# Autodesk Inventor assembly: 18659_pack_assembly
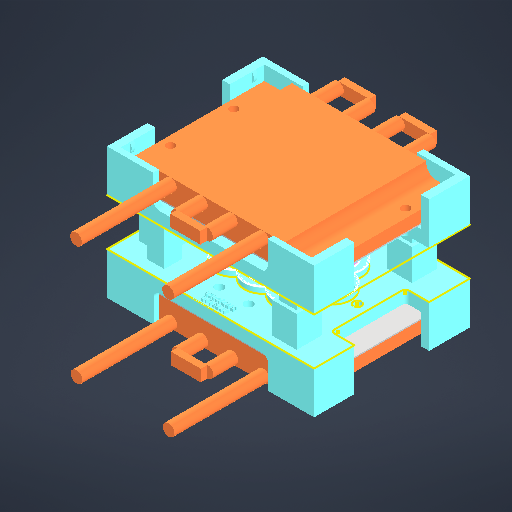
[picture p0: Inventor's stored thumbnail of the model, 512x512]
Saved by Autodesk Inventor 2026.2 (Build 302298000, 298)
## iProperties
Created: 2026-07-18
Part Number: 18659_pack_assembly
Document SubType Name: Assembly
Designer: cbast
Author: cbast
## Documents named in this file (5)
- C:\Users\cbast\OneDrive\Documents\GitHub\Smart-Pack-for-Advanced-Research-and-Control\variations\Camden\V0.2.2\hardware\18650_Pack_CAD\18659_pack_assembly.iam
- C:\Users\cbast\OneDrive\Documents\GitHub\Smart-Pack-for-Advanced-Research-and-Control\variations\Camden\V0.2.2\hardware\18650_Pack_CAD\Pillars_Cellcase_18650.ipt
- C:\Users\cbast\OneDrive\Documents\GitHub\Smart-Pack-for-Advanced-Research-and-Control\variations\Camden\V0.2.2\hardware\18650_Pack_CAD\18650_cell.ipt
- C:\Users\cbast\OneDrive\Documents\GitHub\Smart-Pack-for-Advanced-Research-and-Control\variations\Camden\V0.2.2\hardware\18650_Pack_CAD\thermal_pad.ipt
- C:\Users\cbast\OneDrive\Documents\GitHub\Smart-Pack-for-Advanced-Research-and-Control\variations\Camden\V0.2.2\hardware\18650_Pack_CAD\cooling plate.ipt
## Components (16 placed, 4 different names)
1. Pillars_Cellcase_18650:1 — Mate:1, Mate:2, Flush:1, Flush:2, Mate:3, Mate:4, Mate:5, Mate:6, Mate:7, Mate:8, Mate:9, Mate:10, Mate:11, Mate:12, Mate:14, Mate:15
2. Pillars_Cellcase_18650:2 — Mate:1, Mate:2, Flush:1, Flush:2, Mate:17, Mate:18
3. 18650_cell:1 — Mate:12, Flush:9, Flush:10
4. 18650_cell:2 — Mate:11, Flush:8, Flush:9
5. 18650_cell:3 — Mate:10, Flush:3
6. 18650_cell:4 — Mate:9, Flush:7, Flush:8
7. 18650_cell:5 — Mate:8, Flush:5, Flush:6, Mate:13, Mate:16
8. 18650_cell:6 — Mate:7, Flush:10, Flush:11
9. 18650_cell:7 — Mate:5, Flush:6, Flush:7
10. 18650_cell:8 — Mate:4, Flush:3, Flush:4
11. 18650_cell:9 — Mate:3, Flush:4, Flush:5
12. 18650_cell:10 — Mate:6, Flush:11
13. thermal_pad:1 — Mate:13, Mate:14, Mate:15, Mate:20, Flush:14, Flush:15
14. thermal_pad:2 — Mate:16, Mate:17, Mate:18, Mate:19, Flush:12, Flush:13
15. cooling plate:1 — Mate:19, Flush:12, Flush:13
16. cooling plate:2 — Mate:20, Flush:14, Flush:15
## Relationships (35: Mate 20, Flush 15)
- Mate:1: Pillars_Cellcase_18650:1 ↔ Pillars_Cellcase_18650:2
- Mate:2: Pillars_Cellcase_18650:1 ↔ Pillars_Cellcase_18650:2
- Flush:1: Pillars_Cellcase_18650:1 ↔ Pillars_Cellcase_18650:2
- Flush:2: Pillars_Cellcase_18650:1 ↔ Pillars_Cellcase_18650:2
- Mate:3: Pillars_Cellcase_18650:1 ↔ 18650_cell:9
- Mate:4: Pillars_Cellcase_18650:1 ↔ 18650_cell:8
- Mate:5: Pillars_Cellcase_18650:1 ↔ 18650_cell:7
- Mate:6: Pillars_Cellcase_18650:1 ↔ 18650_cell:10
- Mate:7: Pillars_Cellcase_18650:1 ↔ 18650_cell:6
- Mate:8: Pillars_Cellcase_18650:1 ↔ 18650_cell:5
- Mate:9: Pillars_Cellcase_18650:1 ↔ 18650_cell:4
- Mate:10: Pillars_Cellcase_18650:1 ↔ 18650_cell:3
- Mate:11: Pillars_Cellcase_18650:1 ↔ 18650_cell:2
- Mate:12: Pillars_Cellcase_18650:1 ↔ 18650_cell:1
- Flush:3: 18650_cell:3 ↔ 18650_cell:8
- Flush:4: 18650_cell:8 ↔ 18650_cell:9
- Flush:5: 18650_cell:5 ↔ 18650_cell:9
- Flush:6: 18650_cell:5 ↔ 18650_cell:7
- Flush:7: 18650_cell:4 ↔ 18650_cell:7
- Flush:8: 18650_cell:2 ↔ 18650_cell:4
- Flush:9: 18650_cell:1 ↔ 18650_cell:2
- Flush:10: 18650_cell:1 ↔ 18650_cell:6
- Flush:11: 18650_cell:6 ↔ 18650_cell:10
- Mate:13: 18650_cell:5 ↔ thermal_pad:1
- Mate:14: Pillars_Cellcase_18650:1 ↔ thermal_pad:1
- Mate:15: Pillars_Cellcase_18650:1 ↔ thermal_pad:1
- Mate:16: 18650_cell:5 ↔ thermal_pad:2
- Mate:17: Pillars_Cellcase_18650:2 ↔ thermal_pad:2
- Mate:18: Pillars_Cellcase_18650:2 ↔ thermal_pad:2
- Mate:19: thermal_pad:2 ↔ cooling plate:1
- Flush:12: thermal_pad:2 ↔ cooling plate:1
- Flush:13: thermal_pad:2 ↔ cooling plate:1
- Mate:20: thermal_pad:1 ↔ cooling plate:2
- Flush:14: thermal_pad:1 ↔ cooling plate:2
- Flush:15: thermal_pad:1 ↔ cooling plate:2
